# Autodesk Inventor assembly: Mecanum Right With Roller 1764
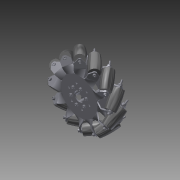
[picture p0: Inventor's stored thumbnail of the model, 180x180]
Saved by Autodesk Inventor 2011 (Build 150239000, 239)
## iProperties
Created: 2011-01-14
Part Number: Mecanum Right With Roller 1764
Document SubType Name: Assembly
Designer: dfranz
Translation Standard: STEP AP203
FileName: //Amserv/amserver/AndyMark/Products/Wheel Mecanum/8 Mecanum Wheel/8 mecanum right with roller.stp
PreProcessor: Unknown
PostProcessor: Build: 239, Release: 2011 RTM - Date: Wed 02/17/2010
Sent Units: millimeter
Uncertainty: 0.001
Author: dfranz
## Documents named in this file (9)
- R:\2010-2011\CAD\Frame 1764\Drive Train 1764\Wheels 1764\Mecanum Wheel 1764\Mecanum Right 1764\Mecanum Right With Roller 1764.iam
- R:\2010-2011\CAD\Frame 1764\Drive Train 1764\Wheels 1764\Mecanum Wheel 1764\Mecanum Right 1764\Washer0 1764.ipt
- R:\2010-2011\CAD\Frame 1764\Drive Train 1764\Wheels 1764\Mecanum Wheel 1764\Mecanum Right 1764\#10 LockNut1 1764.ipt
- R:\2010-2011\CAD\Frame 1764\Drive Train 1764\Wheels 1764\Mecanum Wheel 1764\Mecanum Right 1764\MBC Bushing MU04TH4 1764.ipt
- R:\2010-2011\CAD\Frame 1764\Drive Train 1764\Wheels 1764\Mecanum Wheel 1764\Mecanum Right 1764\Mid Roller III2 1764.ipt
- R:\2010-2011\CAD\Frame 1764\Drive Train 1764\Wheels 1764\Mecanum Wheel 1764\Mecanum Right 1764\SHCS 10-32x3_SHCS 10-32x4 1764.ipt
- R:\2010-2011\CAD\Frame 1764\Drive Train 1764\Wheels 1764\Mecanum Wheel 1764\Mecanum Right 1764\Middle Axle3 1764.ipt
- R:\2010-2011\CAD\Frame 1764\Drive Train 1764\Wheels 1764\Mecanum Wheel 1764\Mecanum Right 1764\Spacer AA 1764.ipt
- R:\2010-2011\CAD\Frame 1764\Drive Train 1764\Wheels 1764\Mecanum Wheel 1764\Mecanum Right 1764\8 Mecanum Plate Right 1764.ipt
## Components (117 placed, 8 different names)
1. Washer0 1764:1 — Insert:77, Insert:78
2. Washer0 1764:2 — Insert:63, Insert:64
3. Washer0 1764:3 — Insert:24, Insert:25
4. Washer0 1764:4 — Insert:16, Insert:17
5. Washer0 1764:5 — Insert:46, Insert:47, Insert:50
6. Washer0 1764:6 — Mate:4
7. Washer0 1764:7 — Insert:95, Insert:96, Insert:97
8. Washer0 1764:8 — Insert:85, Insert:86
9. Washer0 1764:9 — Insert:13, Insert:14, Insert:15
10. Washer0 1764:10 — Insert:70, Insert:71
11. Washer0 1764:11 — Insert:55, Insert:56
12. Washer0 1764:12 — Insert:40, Insert:41
13. Washer0 1764:13 — Insert:48, Insert:49
14. Washer0 1764:14 — Insert:52, Insert:53, Insert:54
15. Washer0 1764:15 — Mate:5, Mate:6, Mate:7, Mate:8
16. Washer0 1764:16 — Insert:30, Insert:31, Insert:34
17. Washer0 1764:17 — Insert:61, Insert:62
18. Washer0 1764:18 — Insert:68, Insert:69, Insert:72
19. Washer0 1764:19 — Insert:87, Insert:88
20. Washer0 1764:20 — Insert:32, Insert:33
21. Washer0 1764:21 — Insert:93, Insert:94
22. Washer0 1764:22 — Insert:79, Insert:80
23. Washer0 1764:23 — Insert:22, Insert:23
24. Washer0 1764:24 — Insert:38, Insert:39
25. #10 LockNut1 1764:1 — Insert:98
26. #10 LockNut1 1764:2 — Insert:43
27. #10 LockNut1 1764:3 — Insert:90
28. #10 LockNut1 1764:4 — Insert:66
29. #10 LockNut1 1764:5 — Insert:27
30. #10 LockNut1 1764:6 — Insert:110
31. #10 LockNut1 1764:7 — Insert:82
32. #10 LockNut1 1764:8 — Insert:58
33. #10 LockNut1 1764:9 — Insert:107
34. #10 LockNut1 1764:10 — Insert:35
35. #10 LockNut1 1764:11 — Insert:19
36. #10 LockNut1 1764:12 — Insert:3
37. #10 LockNut1 1764:13 — Insert:108
38. #10 LockNut1 1764:14 — Insert:109
39. #10 LockNut1 1764:15 — Insert:105
40. #10 LockNut1 1764:16 — Insert:51
41. #10 LockNut1 1764:17 — Insert:74
42. #10 LockNut1 1764:18 — Insert:106
43. MBC Bushing MU04TH4 1764:1 — Insert:31
44. MBC Bushing MU04TH4 1764:2 — Insert:17
45. MBC Bushing MU04TH4 1764:3 — Insert:96
46. MBC Bushing MU04TH4 1764:4 — Insert:94
47. MBC Bushing MU04TH4 1764:5 — Insert:23, Insert:26
48. MBC Bushing MU04TH4 1764:6 — Mate:7, Mate:8
49. MBC Bushing MU04TH4 1764:7 — Insert:39, Insert:42
50. MBC Bushing MU04TH4 1764:8 — Insert:47
51. MBC Bushing MU04TH4 1764:9 — Insert:78, Insert:81
52. MBC Bushing MU04TH4 1764:10 — Insert:80
53. MBC Bushing MU04TH4 1764:11 — Insert:86, Insert:89
54. MBC Bushing MU04TH4 1764:12 — Insert:88
55. MBC Bushing MU04TH4 1764:13 — Insert:25
56. MBC Bushing MU04TH4 1764:14 — Insert:71
57. MBC Bushing MU04TH4 1764:15 — Insert:56
58. MBC Bushing MU04TH4 1764:16 — Mate:11, Mate:12, Insert:4
59. MBC Bushing MU04TH4 1764:17 — Insert:41
60. MBC Bushing MU04TH4 1764:18 — Insert:62, Insert:65
61. MBC Bushing MU04TH4 1764:19 — Insert:64
62. MBC Bushing MU04TH4 1764:20 — Insert:15, Insert:18
63. MBC Bushing MU04TH4 1764:21 — Insert:33
64. MBC Bushing MU04TH4 1764:22 — Insert:54, Insert:57
65. MBC Bushing MU04TH4 1764:23 — Insert:69, Insert:73
66. MBC Bushing MU04TH4 1764:24 — Insert:49
67. Mid Roller III2 1764:1 — Insert:89
68. Mid Roller III2 1764:2 — Insert:81
69. Mid Roller III2 1764:3 — Insert:57
70. Mid Roller III2 1764:4 — Insert:18
71. Mid Roller III2 1764:5 — Insert:50
72. Mid Roller III2 1764:6 — Insert:4
73. Mid Roller III2 1764:7 — Insert:26
74. Mid Roller III2 1764:8 — Insert:73
75. Mid Roller III2 1764:9 — Insert:65
76. Mid Roller III2 1764:10 — Insert:34
77. Mid Roller III2 1764:11 — Insert:42
78. Mid Roller III2 1764:12 — Insert:97
79. SHCS 10-32x3_SHCS 10-32x4 1764:1 — Insert:12
80. SHCS 10-32x3_SHCS 10-32x4 1764:2 — Insert:6
81. SHCS 10-32x3_SHCS 10-32x4 1764:3 — Insert:11
82. SHCS 10-32x3_SHCS 10-32x4 1764:4 — Insert:91
83. SHCS 10-32x3_SHCS 10-32x4 1764:5 — Insert:44
84. SHCS 10-32x3_SHCS 10-32x4 1764:6 — Insert:8
85. SHCS 10-32x3_SHCS 10-32x4 1764:7 — Insert:10
86. SHCS 10-32x3_SHCS 10-32x4 1764:8 — Insert:9
87. SHCS 10-32x3_SHCS 10-32x4 1764:9 — Insert:28
88. SHCS 10-32x3_SHCS 10-32x4 1764:10 — Insert:1
89. SHCS 10-32x3_SHCS 10-32x4 1764:11 — Insert:36
90. SHCS 10-32x3_SHCS 10-32x4 1764:12 — Insert:20
91. SHCS 10-32x3_SHCS 10-32x4 1764:13 — Insert:83
92. SHCS 10-32x3_SHCS 10-32x4 1764:14 — Insert:59
93. SHCS 10-32x3_SHCS 10-32x4 1764:15 — Insert:67
94. SHCS 10-32x3_SHCS 10-32x4 1764:16 — Insert:7
95. SHCS 10-32x3_SHCS 10-32x4 1764:17 — Insert:5
96. SHCS 10-32x3_SHCS 10-32x4 1764:18 — Insert:75
97. Middle Axle3 1764:1 — Insert:92, Insert:93, Insert:95
98. Middle Axle3 1764:2 — Insert:60, Insert:61, Insert:63
99. Middle Axle3 1764:3 — Insert:29, Insert:30, Insert:32
100. Middle Axle3 1764:4 — Insert:76, Insert:77, Insert:79
101. Middle Axle3 1764:5 — Insert:72
102. Middle Axle3 1764:6 — Insert:53, Insert:55
103. Middle Axle3 1764:7 — Insert:45, Insert:46, Insert:48
104. Middle Axle3 1764:8 — Insert:14, Insert:16
105. Middle Axle3 1764:9 — Insert:2
106. Middle Axle3 1764:10 — Insert:37, Insert:38, Insert:40
107. Middle Axle3 1764:11 — Insert:84, Insert:85, Insert:87
108. Middle Axle3 1764:12 — Insert:21, Insert:22, Insert:24
109. Spacer AA 1764:1 — Insert:101
110. Spacer AA 1764:2 — Insert:104
111. Spacer AA 1764:3 — Insert:103
112. Spacer AA 1764:4 — Insert:102
113. Spacer AA 1764:5 — Insert:99
114. Spacer AA 1764:6 — Insert:100
115. 8 Mecanum Plate Right 1764:1 — Mate:1, Mate:2, Mate:3, Mate:4, Mate:9, Mate:10, Insert:1, Insert:5, Insert:6, Insert:7, Insert:8, Insert:9, Insert:10, Insert:11, Insert:12, Insert:13, Insert:20, Insert:21, Insert:28, Insert:29, Insert:36, Insert:37, Insert:44, Insert:45, Insert:52, Insert:59, Insert:60, Insert:67, Insert:68, Insert:75, Insert:76, Insert:83, Insert:84, Insert:91, Insert:92, Insert:99, Insert:100, Insert:101, Insert:102, Insert:103, Insert:104
116. 8 Mecanum Plate Right 1764:2 — Mate:1, Mate:2, Mate:3, Mate:5, Mate:6, Insert:3, Insert:19, Insert:27, Insert:35, Insert:43, Insert:51, Insert:58, Insert:66, Insert:70, Insert:74, Insert:82, Insert:90, Insert:98, Insert:105, Insert:106, Insert:107, Insert:108, Insert:109, Insert:110
117. Washer0 1764:25 — Mate:9, Mate:10, Mate:11, Mate:12, Insert:2
## Relationships (122: Insert 110, Mate 12)
- Mate:1: 8 Mecanum Plate Right 1764:1 ↔ 8 Mecanum Plate Right 1764:2
- Mate:2: 8 Mecanum Plate Right 1764:1 ↔ 8 Mecanum Plate Right 1764:2
- Mate:3 (40.64 mm): 8 Mecanum Plate Right 1764:1 ↔ 8 Mecanum Plate Right 1764:2
- Mate:4: Washer0 1764:6 ↔ 8 Mecanum Plate Right 1764:1
- Mate:5: Washer0 1764:15 ↔ 8 Mecanum Plate Right 1764:2
- Mate:6: Washer0 1764:15 ↔ 8 Mecanum Plate Right 1764:2
- Mate:7: Washer0 1764:15 ↔ MBC Bushing MU04TH4 1764:6
- Mate:8: Washer0 1764:15 ↔ MBC Bushing MU04TH4 1764:6
- Mate:9: 8 Mecanum Plate Right 1764:1 ↔ Washer0 1764:25
- Mate:10: 8 Mecanum Plate Right 1764:1 ↔ Washer0 1764:25
- Mate:11: MBC Bushing MU04TH4 1764:16 ↔ Washer0 1764:25
- Mate:12: MBC Bushing MU04TH4 1764:16 ↔ Washer0 1764:25
- Insert:1: SHCS 10-32x3_SHCS 10-32x4 1764:10 ↔ 8 Mecanum Plate Right 1764:1
- Insert:2: Middle Axle3 1764:9 ↔ Washer0 1764:25
- Insert:3: #10 LockNut1 1764:12 ↔ 8 Mecanum Plate Right 1764:2
- Insert:4: MBC Bushing MU04TH4 1764:16 ↔ Mid Roller III2 1764:6
- Insert:5: SHCS 10-32x3_SHCS 10-32x4 1764:17 ↔ 8 Mecanum Plate Right 1764:1
- Insert:6: SHCS 10-32x3_SHCS 10-32x4 1764:2 ↔ 8 Mecanum Plate Right 1764:1
- Insert:7: SHCS 10-32x3_SHCS 10-32x4 1764:16 ↔ 8 Mecanum Plate Right 1764:1
- Insert:8: SHCS 10-32x3_SHCS 10-32x4 1764:6 ↔ 8 Mecanum Plate Right 1764:1
- Insert:9: SHCS 10-32x3_SHCS 10-32x4 1764:8 ↔ 8 Mecanum Plate Right 1764:1
- Insert:10: SHCS 10-32x3_SHCS 10-32x4 1764:7 ↔ 8 Mecanum Plate Right 1764:1
- Insert:11: SHCS 10-32x3_SHCS 10-32x4 1764:3 ↔ 8 Mecanum Plate Right 1764:1
- Insert:12: SHCS 10-32x3_SHCS 10-32x4 1764:1 ↔ 8 Mecanum Plate Right 1764:1
- Insert:13: Washer0 1764:9 ↔ 8 Mecanum Plate Right 1764:1
- Insert:14: Washer0 1764:9 ↔ Middle Axle3 1764:8
- Insert:15: Washer0 1764:9 ↔ MBC Bushing MU04TH4 1764:20
- Insert:16: Washer0 1764:4 ↔ Middle Axle3 1764:8
- Insert:17: Washer0 1764:4 ↔ MBC Bushing MU04TH4 1764:2
- Insert:18: MBC Bushing MU04TH4 1764:20 ↔ Mid Roller III2 1764:4
- Insert:19: #10 LockNut1 1764:11 ↔ 8 Mecanum Plate Right 1764:2
- Insert:20: SHCS 10-32x3_SHCS 10-32x4 1764:12 ↔ 8 Mecanum Plate Right 1764:1
- Insert:21: Middle Axle3 1764:12 ↔ 8 Mecanum Plate Right 1764:1
- Insert:22: Washer0 1764:23 ↔ Middle Axle3 1764:12
- Insert:23: Washer0 1764:23 ↔ MBC Bushing MU04TH4 1764:5
- Insert:24: Washer0 1764:3 ↔ Middle Axle3 1764:12
- Insert:25: Washer0 1764:3 ↔ MBC Bushing MU04TH4 1764:13
- Insert:26: MBC Bushing MU04TH4 1764:5 ↔ Mid Roller III2 1764:7
- Insert:27: #10 LockNut1 1764:5 ↔ 8 Mecanum Plate Right 1764:2
- Insert:28: SHCS 10-32x3_SHCS 10-32x4 1764:9 ↔ 8 Mecanum Plate Right 1764:1
- Insert:29: Middle Axle3 1764:3 ↔ 8 Mecanum Plate Right 1764:1
- Insert:30: Washer0 1764:16 ↔ Middle Axle3 1764:3
- Insert:31: Washer0 1764:16 ↔ MBC Bushing MU04TH4 1764:1
- Insert:32: Washer0 1764:20 ↔ Middle Axle3 1764:3
- Insert:33: Washer0 1764:20 ↔ MBC Bushing MU04TH4 1764:21
- Insert:34: Washer0 1764:16 ↔ Mid Roller III2 1764:10
- Insert:35: #10 LockNut1 1764:10 ↔ 8 Mecanum Plate Right 1764:2
- Insert:36: SHCS 10-32x3_SHCS 10-32x4 1764:11 ↔ 8 Mecanum Plate Right 1764:1
- Insert:37: Middle Axle3 1764:10 ↔ 8 Mecanum Plate Right 1764:1
- Insert:38: Washer0 1764:24 ↔ Middle Axle3 1764:10
- Insert:39: Washer0 1764:24 ↔ MBC Bushing MU04TH4 1764:7
- Insert:40: Washer0 1764:12 ↔ Middle Axle3 1764:10
- Insert:41: Washer0 1764:12 ↔ MBC Bushing MU04TH4 1764:17
- Insert:42: MBC Bushing MU04TH4 1764:7 ↔ Mid Roller III2 1764:11
- Insert:43: #10 LockNut1 1764:2 ↔ 8 Mecanum Plate Right 1764:2
- Insert:44: SHCS 10-32x3_SHCS 10-32x4 1764:5 ↔ 8 Mecanum Plate Right 1764:1
- Insert:45: Middle Axle3 1764:7 ↔ 8 Mecanum Plate Right 1764:1
- Insert:46: Washer0 1764:5 ↔ Middle Axle3 1764:7
- Insert:47: Washer0 1764:5 ↔ MBC Bushing MU04TH4 1764:8
- Insert:48: Washer0 1764:13 ↔ Middle Axle3 1764:7
- Insert:49: Washer0 1764:13 ↔ MBC Bushing MU04TH4 1764:24
- Insert:50: Washer0 1764:5 ↔ Mid Roller III2 1764:5
- Insert:51: #10 LockNut1 1764:16 ↔ 8 Mecanum Plate Right 1764:2
- Insert:52: Washer0 1764:14 ↔ 8 Mecanum Plate Right 1764:1
- Insert:53: Washer0 1764:14 ↔ Middle Axle3 1764:6
- Insert:54: Washer0 1764:14 ↔ MBC Bushing MU04TH4 1764:22
- Insert:55: Washer0 1764:11 ↔ Middle Axle3 1764:6
- Insert:56: Washer0 1764:11 ↔ MBC Bushing MU04TH4 1764:15
- Insert:57: MBC Bushing MU04TH4 1764:22 ↔ Mid Roller III2 1764:3
- Insert:58: #10 LockNut1 1764:8 ↔ 8 Mecanum Plate Right 1764:2
- Insert:59: SHCS 10-32x3_SHCS 10-32x4 1764:14 ↔ 8 Mecanum Plate Right 1764:1
- Insert:60: Middle Axle3 1764:2 ↔ 8 Mecanum Plate Right 1764:1
- Insert:61: Washer0 1764:17 ↔ Middle Axle3 1764:2
- Insert:62: Washer0 1764:17 ↔ MBC Bushing MU04TH4 1764:18
- Insert:63: Washer0 1764:2 ↔ Middle Axle3 1764:2
- Insert:64: Washer0 1764:2 ↔ MBC Bushing MU04TH4 1764:19
- Insert:65: MBC Bushing MU04TH4 1764:18 ↔ Mid Roller III2 1764:9
- Insert:66: #10 LockNut1 1764:4 ↔ 8 Mecanum Plate Right 1764:2
- Insert:67: SHCS 10-32x3_SHCS 10-32x4 1764:15 ↔ 8 Mecanum Plate Right 1764:1
- Insert:68: Washer0 1764:18 ↔ 8 Mecanum Plate Right 1764:1
- Insert:69: Washer0 1764:18 ↔ MBC Bushing MU04TH4 1764:23
- Insert:70: Washer0 1764:10 ↔ 8 Mecanum Plate Right 1764:2
- Insert:71: Washer0 1764:10 ↔ MBC Bushing MU04TH4 1764:14
- Insert:72: Washer0 1764:18 ↔ Middle Axle3 1764:5
- Insert:73: MBC Bushing MU04TH4 1764:23 ↔ Mid Roller III2 1764:8
- Insert:74: #10 LockNut1 1764:17 ↔ 8 Mecanum Plate Right 1764:2
- Insert:75: SHCS 10-32x3_SHCS 10-32x4 1764:18 ↔ 8 Mecanum Plate Right 1764:1
- Insert:76: Middle Axle3 1764:4 ↔ 8 Mecanum Plate Right 1764:1
- Insert:77: Washer0 1764:1 ↔ Middle Axle3 1764:4
- Insert:78: Washer0 1764:1 ↔ MBC Bushing MU04TH4 1764:9
- Insert:79: Washer0 1764:22 ↔ Middle Axle3 1764:4
- Insert:80: Washer0 1764:22 ↔ MBC Bushing MU04TH4 1764:10
- Insert:81: MBC Bushing MU04TH4 1764:9 ↔ Mid Roller III2 1764:2
- Insert:82: #10 LockNut1 1764:7 ↔ 8 Mecanum Plate Right 1764:2
- Insert:83: SHCS 10-32x3_SHCS 10-32x4 1764:13 ↔ 8 Mecanum Plate Right 1764:1
- Insert:84: Middle Axle3 1764:11 ↔ 8 Mecanum Plate Right 1764:1
- Insert:85: Washer0 1764:8 ↔ Middle Axle3 1764:11
- Insert:86: Washer0 1764:8 ↔ MBC Bushing MU04TH4 1764:11
- Insert:87: Washer0 1764:19 ↔ Middle Axle3 1764:11
- Insert:88: Washer0 1764:19 ↔ MBC Bushing MU04TH4 1764:12
- Insert:89: MBC Bushing MU04TH4 1764:11 ↔ Mid Roller III2 1764:1
- Insert:90: #10 LockNut1 1764:3 ↔ 8 Mecanum Plate Right 1764:2
- Insert:91: SHCS 10-32x3_SHCS 10-32x4 1764:4 ↔ 8 Mecanum Plate Right 1764:1
- Insert:92: Middle Axle3 1764:1 ↔ 8 Mecanum Plate Right 1764:1
- Insert:93: Washer0 1764:21 ↔ Middle Axle3 1764:1
- Insert:94: Washer0 1764:21 ↔ MBC Bushing MU04TH4 1764:4
- Insert:95: Washer0 1764:7 ↔ Middle Axle3 1764:1
- Insert:96: Washer0 1764:7 ↔ MBC Bushing MU04TH4 1764:3
- Insert:97: Washer0 1764:7 ↔ Mid Roller III2 1764:12
- Insert:98: #10 LockNut1 1764:1 ↔ 8 Mecanum Plate Right 1764:2
- Insert:99: Spacer AA 1764:5 ↔ 8 Mecanum Plate Right 1764:1
- Insert:100: Spacer AA 1764:6 ↔ 8 Mecanum Plate Right 1764:1
- Insert:101: Spacer AA 1764:1 ↔ 8 Mecanum Plate Right 1764:1
- Insert:102: Spacer AA 1764:4 ↔ 8 Mecanum Plate Right 1764:1
- Insert:103: Spacer AA 1764:3 ↔ 8 Mecanum Plate Right 1764:1
- Insert:104: Spacer AA 1764:2 ↔ 8 Mecanum Plate Right 1764:1
- Insert:105: #10 LockNut1 1764:15 ↔ 8 Mecanum Plate Right 1764:2
- Insert:106: #10 LockNut1 1764:18 ↔ 8 Mecanum Plate Right 1764:2
- Insert:107: #10 LockNut1 1764:9 ↔ 8 Mecanum Plate Right 1764:2
- Insert:108: #10 LockNut1 1764:13 ↔ 8 Mecanum Plate Right 1764:2
- Insert:109: #10 LockNut1 1764:14 ↔ 8 Mecanum Plate Right 1764:2
- Insert:110: #10 LockNut1 1764:6 ↔ 8 Mecanum Plate Right 1764:2
